# Autodesk Inventor assembly: Z
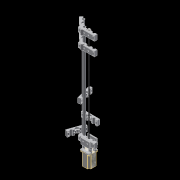
[picture p0: Inventor's stored thumbnail of the model, 180x180]
Saved by Autodesk Inventor 2016 (Build 200138000, 138)
## iProperties
Created: 2017-07-13
Part Number: Z
Document SubType Name: Assembly
Designer: ludwi
Author: ludwi
## Documents named in this file (8)
- H:\MARQ\3D\AXIS_DEV_EDT_V3\Y.iam
- H:\MARQ\3D\AXIS_DEV_EDT_V3\AXB.ipt
- C:\Users\ludwi\OneDrive\Documentos\Inventor\Content Center Files\R2016\en-US\DIN BEARING(1)\DIN 625 SKF - SKF 626.ipt
- C:\Users\ludwi\OneDrive\Documentos\Inventor\Content Center Files\R2016\en-US\DIN 935\DIN 935 T1 - M6 x 1 x 10.ipt
- H:\MARQ\3D\AXIS_DEV_EDT_V3\NEMA23.ipt
- H:\MARQ\3D\AXIS_DEV_EDT_V3\MSUP.ipt
- H:\MARQ\3D\AXIS_DEV_EDT_V3\TuboEstructura.ipt
- H:\MARQ\3D\AXIS_DEV_EDT_V3\M6SM.ipt
## Components (18 placed, 7 different names)
1. AXB:1 — Insert:9, Insert:19
2. AXB:2 — Insert:16, Insert:17
3. AXB:3 — Insert:10
4. AXB:4 — Insert:18
5. DIN 625 SKF SKF 626:1 — Insert:9, Mate:6
6. DIN 625 SKF SKF 626:2 — Insert:10, Mate:4
7. DIN 935 M6:1 — Mate:4
8. DIN 935 M6:2 — Mate:6
9. NEMA23:1 — Flush:2, Insert:13, Insert:14, Insert:20
10. MSUP:1 — Flush:2
11. MSUP:2 — Insert:13, Insert:14
12. TuboEstructura:1 — Insert:16, Insert:18, Mate:7, Mate:12
13. TuboEstructura:2 — Insert:17, Insert:19, Mate:8, Mate:9, Mate:13
14. M6SM:1 — Insert:20
15. AXB:5 — Mate:7, Mate:8, Mate:9
16. AXB:6
17. AXB:9 — Mate:13
18. AXB:10 — Mate:12
## Relationships (17: Insert 9, Mate 7, Flush 1)
- Insert:9: AXB:1 ↔ DIN 625 SKF SKF 626:1
- Insert:10: AXB:3 ↔ DIN 625 SKF SKF 626:2
- Mate:4: DIN 625 SKF SKF 626:2 ↔ DIN 935 M6:1
- Mate:6: DIN 625 SKF SKF 626:1 ↔ DIN 935 M6:2
- Flush:2: NEMA23:1 ↔ MSUP:1
- Insert:13: NEMA23:1 ↔ MSUP:2
- Insert:14: NEMA23:1 ↔ MSUP:2
- Insert:16: AXB:2 ↔ TuboEstructura:1
- Insert:17: AXB:2 ↔ TuboEstructura:2
- Insert:18: AXB:4 ↔ TuboEstructura:1
- Insert:19: AXB:1 ↔ TuboEstructura:2
- Insert:20: NEMA23:1 ↔ M6SM:1
- Mate:7: TuboEstructura:1 ↔ AXB:5
- Mate:8: TuboEstructura:2 ↔ AXB:5
- Mate:9: TuboEstructura:2 ↔ AXB:5
- Mate:12: TuboEstructura:1 ↔ AXB:10
- Mate:13: TuboEstructura:2 ↔ AXB:9
